# Autodesk Inventor assembly: Ground_Tracker
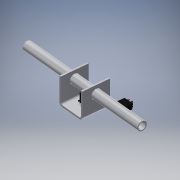
[picture p0: Inventor's stored thumbnail of the model, 180x180]
Saved by Autodesk Inventor 2018 (Build 220112000, 112)
## iProperties
Created: 2018-09-27
Part Number: Ground_Tracker
Document SubType Name: Assembly
Designer: Bradley
Author: Bradley
## Documents named in this file (6)
- C:\Users\Bradley\Documents\CougsInSpace\CougSat1-Hardware\CougSat1-GroundStation\CADModel\Native\Ground_Tracker.iam
- C:\Users\Bradley\Documents\CougsInSpace\CougSat1-Hardware\CougSat1-GroundStation\CADModel\Native\Ground_Tracker_TripodMount.ipt
- C:\Users\Bradley\Documents\CougsInSpace\CougSat1-Hardware\CougSat1-GroundStation\CADModel\Native\Ground_Tracker_Bearing.ipt
- C:\Users\Bradley\Documents\CougsInSpace\CougSat1-Hardware\CougSat1-GroundStation\CADModel\Native\Ground_Tracker_CrossTube.ipt
- C:\Users\Bradley\Documents\CougsInSpace\Resources\ComponentModels\Hardware\Coupler_ServoHub.ipt
- C:\Users\Bradley\Documents\CougsInSpace\Resources\ComponentModels\Electronics\Servo_Standard.ipt
## Components (6 placed, 5 different names)
1. Ground_Tracker_TripodMount:1 — Insert:1, Insert:2, Insert:3
2. Ground_Tracker_Bearing:1 — Insert:1, Mate:1, Flush:1, Mate:2
3. Ground_Tracker_CrossTube:1 — Mate:1, Flush:1
4. Coupler_ServoHub:1 — Insert:2, Insert:3, Insert:4
5. Servo_Standard:1 — Insert:4
6. Servo_Standard:2 — Mate:2
## Relationships (7: Insert 4, Mate 2, Flush 1)
- Insert:1: Ground_Tracker_TripodMount:1 ↔ Ground_Tracker_Bearing:1
- Mate:1: Ground_Tracker_Bearing:1 ↔ Ground_Tracker_CrossTube:1
- Flush:1: Ground_Tracker_Bearing:1 ↔ Ground_Tracker_CrossTube:1
- Insert:2: Ground_Tracker_TripodMount:1 ↔ Coupler_ServoHub:1
- Insert:3: Ground_Tracker_TripodMount:1 ↔ Coupler_ServoHub:1
- Insert:4: Coupler_ServoHub:1 ↔ Servo_Standard:1
- Mate:2: Ground_Tracker_Bearing:1 ↔ Servo_Standard:2
